# Autodesk Inventor assembly: v2-VersaPlanetary-1stage-with-775pro-20161031
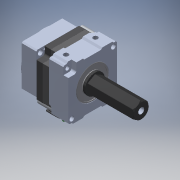
[picture p0: Inventor's stored thumbnail of the model, 180x180]
Saved by Autodesk Inventor 2018 (Build 220112000, 112)
## iProperties
Created: 2016-10-31
Part Number: v2-VersaPlanetary-1stage-with-775pro-20161031
Description: STEP AP214
Document SubType Name: Assembly
Designer: snipe
Sending System: SolidWorks 2016
Preprocessor: SwSTEP 2.0
Title: 217-4973_1stage_775pro.STEP
Revision Number: ANY
## Documents named in this file (9)
- E:\50000skater\Assets\VPlanRingGear.iam
- E:\50000skater\Assets\Resources\217-2625-026 Rev1.ipt
- E:\50000skater\Assets\Resources\217-2742-001 Rev4.ipt
- E:\50000skater\Assets\Resources\217-2625-017 Rev1_9714K61.ipt
- E:\50000skater\Assets\Resources\217-2625-003 Rev1.ipt
- E:\50000skater\Assets\Resources\217-2625-018 Rev1_98541A410.ipt
- E:\50000skater\Assets\Resources\217-2820 Rev1_Public.iam
- E:\50000skater\Assets\Resources\217-2816-001 Rev1.ipt
- E:\50000skater\Assets\VPlanIntegEnc.iam
## Components (9 placed, 9 different names)
1. 217-2625-026 Rev1_1 — Mate:1, Flush:1, Mate:2, Mate:3, Mate:4, Mate:5, Flush:2, Mate:9, Mate:10, Mate:11, Flush:3, Mate:13, Mate:14, Flush:4, Flush:5, Mate:17, Mate:18
2. 217-2742-001 Rev4_2 — Mate:5, Flush:2, Mate:8
3. 217-2742-001 Rev4_3 — Mate:1, Flush:1, Mate:6, Mate:7
4. 217-2625-017 Rev1_9714K61_4 — Mate:2, Mate:3, Mate:4
5. 217-2625-003 Rev1_5 — Mate:6, Mate:7, Mate:9, Mate:10, Mate:12
6. 217-2625-018 Rev1_98541A410_6 — Mate:8, Mate:11, Flush:3
7. 217-2820 Rev1_Public_16 [sub-assembly] — Mate:16, Mate:17, Mate:18
8. 217-2816-001 Rev1_17 — Mate:15, Flush:4, Flush:5
9. VPlanIntegEnc:1 [sub-assembly] — Mate:12, Mate:13, Mate:14, Mate:15, Mate:16
## Relationships (23: Mate 18, Flush 5)
- Mate:1: 217-2625-026 Rev1_1 ↔ 217-2742-001 Rev4_3
- Flush:1: 217-2625-026 Rev1_1 ↔ 217-2742-001 Rev4_3
- Mate:2: 217-2625-026 Rev1_1 ↔ 217-2625-017 Rev1_9714K61_4
- Mate:3: 217-2625-026 Rev1_1 ↔ 217-2625-017 Rev1_9714K61_4
- Mate:4: 217-2625-026 Rev1_1 ↔ 217-2625-017 Rev1_9714K61_4
- Mate:5: 217-2625-026 Rev1_1 ↔ 217-2742-001 Rev4_2
- Flush:2: 217-2625-026 Rev1_1 ↔ 217-2742-001 Rev4_2
- Mate:6: 217-2742-001 Rev4_3 ↔ 217-2625-003 Rev1_5
- Mate:7: 217-2742-001 Rev4_3 ↔ 217-2625-003 Rev1_5
- Mate:8: 217-2742-001 Rev4_2 ↔ 217-2625-018 Rev1_98541A410_6
- Mate:9: 217-2625-026 Rev1_1 ↔ 217-2625-003 Rev1_5
- Mate:10: 217-2625-026 Rev1_1 ↔ 217-2625-003 Rev1_5
- Mate:11: 217-2625-026 Rev1_1 ↔ 217-2625-018 Rev1_98541A410_6
- Flush:3: 217-2625-026 Rev1_1 ↔ 217-2625-018 Rev1_98541A410_6
- Mate:12: 217-2625-003 Rev1_5 ↔ VPlanIntegEnc:1
- Mate:13: 217-2625-026 Rev1_1 ↔ VPlanIntegEnc:1
- Mate:14: 217-2625-026 Rev1_1 ↔ VPlanIntegEnc:1
- Mate:15: 217-2816-001 Rev1_17 ↔ VPlanIntegEnc:1
- Flush:4: 217-2625-026 Rev1_1 ↔ 217-2816-001 Rev1_17
- Flush:5: 217-2625-026 Rev1_1 ↔ 217-2816-001 Rev1_17
- Mate:16: 217-2820 Rev1_Public_16 ↔ VPlanIntegEnc:1
- Mate:17: 217-2625-026 Rev1_1 ↔ 217-2820 Rev1_Public_16
- Mate:18: 217-2625-026 Rev1_1 ↔ 217-2820 Rev1_Public_16
